# Autodesk Inventor assembly: Test Cut
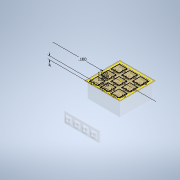
[picture p0: Inventor's stored thumbnail of the model, 180x180]
Saved by Autodesk Inventor 2022 (Build 260153000, 153)
## iProperties
Created: 2022-03-04
Part Number: Test Cut
Document SubType Name: Assembly
Designer: Nathan Griffith
Author: Nathan Griffith
## Documents named in this file (5)
- C:\Users\Nathan Griffith\Documents\Inventor\Eric's Keyboard\Eric60percentkeyboard\Inventor\Test Cut.iam
- C:\Users\Nathan Griffith\Documents\Inventor\Eric's Keyboard\Eric60percentkeyboard\Inventor\Holder.iam
- C:\Users\Nathan Griffith\Documents\Inventor\Eric's Keyboard\Eric60percentkeyboard\Inventor\Keycap.ipt
- C:\Users\Nathan Griffith\Documents\Inventor\Eric's Keyboard\Eric60percentkeyboard\Inventor\keycap sepretated\Stock 3x3x1.5.ipt
- C:\Users\Nathan Griffith\Documents\Inventor\Eric's Keyboard\Eric60percentkeyboard\Inventor\keycap sepretated\Template.ipt
## Components (12 placed, 4 different names)
1. Holder:1 [sub-assembly]
2. Stock 3x3x1.5:1 — Flush:1
3. Template:1 — Flush:2, Flush:3, Mate:1, Mate:2, Mate:3
4. Keycap:1 — Mate:1, Mate:2, Mate:3
5. Keycap:2
6. Keycap:3
7. Keycap:4
8. Keycap:5
9. Keycap:6
10. Keycap:7
11. Keycap:8
12. Keycap:9
## Component patterns: (9 elements, first: Keycap:1)
## Relationships (6: Flush 3, Mate 3)
- Flush:1 (-1.27 mm): Stock 3x3x1.5:1
- Flush:2: Template:1
- Flush:3: Template:1
- Mate:1: Template:1 ↔ Keycap:1
- Mate:2: Template:1 ↔ Keycap:1
- Mate:3: Template:1 ↔ Keycap:1
